# Autodesk Inventor assembly: TuppyMkIV Assembly
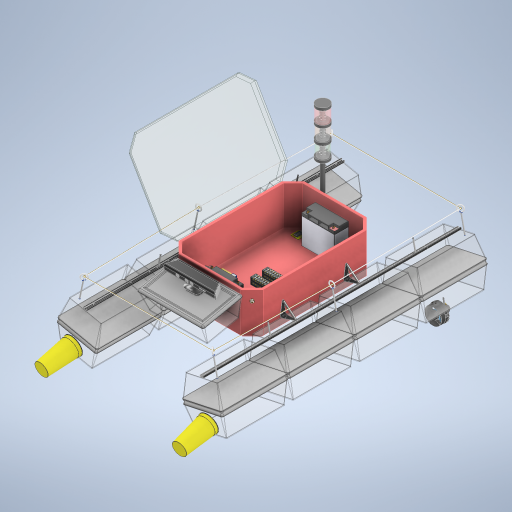
[picture p0: Inventor's stored thumbnail of the model, 512x512]
Saved by Autodesk Inventor 2024 (Build 280153000, 153)
## iProperties
Created: 2023-06-09
Part Number: TuppyMkIV Assembly
Document SubType Name: Assembly
Designer: 18179
Author: 18179
## Documents named in this file (27)
- C:\Users\18179\Desktop\TuppyMkIV\TuppyMkIV Assembly.iam
- C:\Users\18179\Desktop\TuppyMkIV\SmallContainerAssembly.iam
- C:\Users\18179\Desktop\TuppyMkIV\WaterAndBoatLimit.ipt
- C:\Users\18179\Desktop\TuppyMkIV\T200Thruster.ipt
- C:\Users\18179\Desktop\TuppyMkIV\ESC_Assembly.iam
- C:\Users\18179\Desktop\TuppyMkIV\BigContainerLid.ipt
- C:\Users\18179\Desktop\TuppyMkIV\BigContainer.ipt
- C:\Users\18179\Desktop\TuppyMkIV\LightTower.ipt
- C:\Users\18179\Desktop\TuppyMkIV\ProArduino.ipt
- C:\Users\18179\Desktop\TuppyMkIV\RPI\Raspberry Pi 4 Model B.iam
- C:\Users\18179\Downloads\kinect-xbox-360.snapshot.4\Kinect\Kinect.ipt
- C:\Users\18179\Desktop\TuppyMkIV\12Vto5V Converter.ipt
- C:\Users\18179\Desktop\TuppyMkIV\Battery.ipt
- C:\Users\18179\Desktop\TuppyMkIV\CableGland.ipt
- C:\Users\18179\Desktop\TuppyMkIV\RC_Receiver.ipt
- C:\Users\18179\Desktop\TuppyMkIV\EyeBolt.ipt
- C:\Users\18179\Desktop\TuppyMkIV\Hinge.ipt
- C:\Users\18179\Desktop\TuppyMkIV\Hinge_MIR.ipt
- C:\Users\18179\Desktop\TuppyMkIV\Dickey'sBigYellowCup.ipt
- C:\Users\18179\Desktop\TuppyMkIV\C-Channel.ipt
- C:\Users\18179\Desktop\TuppyMkIV\TerminalBlock.ipt
- C:\Users\18179\Desktop\TuppyMkIV\TerminalBlockLid.ipt
- C:\Users\18179\Desktop\TuppyMkIV\Steelbar.ipt
- C:\Users\18179\Desktop\TuppyMkIV\Steelbar_MIR.ipt
- C:\Users\18179\Desktop\TuppyMkIV\C-Channel_7.334in.ipt
- C:\Users\18179\Desktop\TuppyMkIV\TuppyMkIV Assembly\AIP\Cable and Harness\TuppyMkIV Assembly.Harness4.iam
- C:\Users\18179\Desktop\TuppyMkIV\TeeBolt.ipt
## Components (73 placed, 26 different names)
1. WaterAndBoatLimit:1
2. BigContainer:1 — Mate:8, Mate:9, Mate:10, Mate:18, Mate:19, Mate:20, Mate:29, Mate:30, Mate:31, Mate:32, Mate:33, Mate:34, Flush:29, Rotational:1, Mate:36, Mate:37, Mate:38, Mate:39, Mate:45, Mate:51, Mate:52, Mate:53, Mate:54, Mate:55, Mate:56, Mate:57, Flush:36, Flush:37, Mate:58, Mate:59, Mate:60, Mate:63, Mate:64, Flush:45, Mate:75, Mate:76, Angle:1, Angle:2, Angle:3, Mate:98, Mate:103, Mate:104, Mate:105, Mate:106, Mate:107
3. SmallContainerAssembly:1 [sub-assembly] — Flush:1, Flush:4, Flush:5, Mate:1, Flush:13, Flush:14, Mate:81, Mate:82, Tangent:2
4. SmallContainerAssembly:2 [sub-assembly] — Flush:1, Flush:3, Flush:4, Mate:1, Mate:2, Mate:7
5. SmallContainerAssembly:3 [sub-assembly] — Flush:2, Flush:3, Flush:5, Flush:6, Mate:3, Mate:43, Flush:31, Flush:33
6. SmallContainerAssembly:4 [sub-assembly] — Flush:2, Flush:6, Mate:2, Mate:3
7. SmallContainerAssembly:5 [sub-assembly] — Mate:86, Tangent:7, Tangent:8
8. SmallContainerAssembly:6 [sub-assembly] — Mate:7, Mate:8, Mate:10, Mate:66, Flush:43
9. SmallContainerAssembly:7 [sub-assembly] — Flush:13, Flush:14, Mate:84, Tangent:5, Tangent:6, Flush:51, Flush:52, Mate:92
10. SmallContainerAssembly:8 [sub-assembly] — Mate:9, Mate:65, Flush:44, Mate:85, Tangent:13, Tangent:14
11. SmallContainerAssembly:9 [sub-assembly] — Mate:80, Mate:83, Tangent:1
12. SmallContainerAssembly:10 [sub-assembly]
13. SmallContainerAssembly:11 [sub-assembly] — Mate:44, Flush:32, Flush:34
14. SmallContainerAssembly:12 [sub-assembly]
15. SmallContainerAssembly:13 [sub-assembly] — Mate:87, Tangent:9, Tangent:10
16. SmallContainerAssembly:14 [sub-assembly] — Mate:18, Mate:19, Mate:77, Flush:46
17. SmallContainerAssembly:15 [sub-assembly] — Mate:88, Tangent:3, Tangent:4, Mate:93, Flush:53, Flush:54
18. SmallContainerAssembly:16 [sub-assembly] — Mate:20, Mate:78, Mate:79, Mate:89, Tangent:11, Tangent:12
19. ESC_Assembly:1 [sub-assembly] — Mate:29, Mate:31, Mate:33
20. ESC_Assembly:2 [sub-assembly] — Mate:30, Mate:32, Mate:34
21. BigContainerLid:1 — Flush:29, Rotational:1
22. LightTower:1 — Mate:57, Flush:36, Flush:37
23. ProArduino:1 — Mate:36
24. Raspberry Pi 4 Model B:1 [sub-assembly] — Mate:37
25. T200Thruster:1 — Mate:43, Flush:31, Flush:33
26. T200Thruster:2 — Mate:44, Flush:32, Flush:34
27. SmallContainerAssembly:20 [sub-assembly] — Mate:38, Mate:39, Mate:40, Mate:41, Mate:42, Mate:58
28. Kinect:1 — Mate:40, Mate:41, Mate:42
29. 12Vto5V Converter:2 — Mate:45
30. Battery:1 — Mate:104, Mate:106, Flush:56, Flush:59
31. Battery:2 — Mate:105, Mate:107, Flush:55, Mate:108
32. CableGland:1 — Mate:51, Mate:52, Angle:3
33. CableGland:2 — Mate:53, Mate:56, Angle:2
34. CableGland:3 — Mate:54, Mate:55, Angle:1
35. RC_Receiver:1 — Mate:60, Flush:38
36. RC_Receiver:2 — Mate:59, Flush:38
37. Hinge:1 — Mate:63, Mate:69, Mate:70, Mate:109, Mate:111, Mate:112
38. Hinge:2 — Mate:64, Mate:67, Mate:68, Flush:43, Mate:113, Mate:114, Mate:116
39. Hinge:3 — Mate:65, Mate:69, Mate:70, Flush:44, Mate:110
40. Hinge:4 — Mate:66, Mate:67, Mate:68, Mate:115
41. Hinge_MIR:1 — Mate:71, Mate:72, Mate:75, Mate:118, Mate:119, Mate:120
42. Hinge_MIR:2 — Mate:73, Mate:74, Mate:76, Flush:46, Mate:122, Mate:123, Mate:124
43. Hinge_MIR:3 — Mate:71, Mate:72, Mate:78, Mate:79, Mate:117
44. Hinge_MIR:4 — Mate:73, Mate:74, Mate:77, Mate:121
45. Dickey'sBigYellowCup:1 — Mate:81, Mate:82, Tangent:2
46. Dickey'sBigYellowCup:2 — Mate:80, Mate:83, Tangent:1
47. EyeBolt:1 — Mate:88, Tangent:3, Tangent:4
48. EyeBolt:2 — Mate:89, Tangent:11, Tangent:12
49. EyeBolt:3 — Mate:87, Tangent:9, Tangent:10
50. EyeBolt:4 — Mate:86, Tangent:7, Tangent:8
51. EyeBolt:5 — Mate:85, Tangent:13, Tangent:14
52. EyeBolt:6 — Mate:84, Tangent:5, Tangent:6
53. C-Channel:1 — Mate:91, Flush:49, Flush:50, Mate:93, Flush:53, Flush:54, Mate:131, Mate:132, Mate:133, Mate:134
54. C-Channel:2 — Mate:91, Flush:49, Flush:50, Mate:126, Flush:62, Flush:63
55. C-Channel:3 — Mate:90, Flush:47, Flush:48, Flush:51, Flush:52, Mate:92, Mate:127, Mate:128, Mate:129, Mate:130
56. C-Channel:4 — Mate:90, Flush:47, Flush:48, Flush:60, Mate:125, Flush:61
57. TerminalBlock:1 — Mate:94, Mate:95, Mate:96, Mate:97, Flush:58
58. TerminalBlockLid:1 — Mate:94, Mate:95
59. TerminalBlock:2 — Mate:96, Mate:97, Mate:98, Flush:59
60. TerminalBlock:3 — Mate:108, Flush:57
61. TerminalBlockLid:2
62. TerminalBlock:4 — Mate:103
63. Steelbar:1 — Mate:109, Mate:110, Mate:111, Mate:112
64. Steelbar:2 — Mate:113, Mate:114, Mate:115, Mate:116
65. Steelbar_MIR:1 — Mate:117, Mate:118, Mate:119, Mate:120
66. Steelbar_MIR:2 — Mate:121, Mate:122, Mate:123, Mate:124
67. C-Channel_7.334in:1 — Flush:60, Mate:125, Flush:61
68. C-Channel_7.334in:2 — Mate:126, Flush:62, Flush:63
69. Harness4 [sub-assembly]
70. TeeBolt:1 — Mate:131, Mate:132
71. TeeBolt:2 — Mate:133, Mate:134
72. TeeBolt:3 — Mate:129, Mate:130
73. TeeBolt:4 — Mate:127, Mate:128
## Relationships (193: Mate 118, Flush 57, Tangent 14, Angle 3, RevoluteJoint 1)
- Flush:1: SmallContainerAssembly:1 ↔ SmallContainerAssembly:2
- Flush:2: SmallContainerAssembly:3 ↔ SmallContainerAssembly:4
- Flush:3: SmallContainerAssembly:2 ↔ SmallContainerAssembly:3
- Flush:4: SmallContainerAssembly:1 ↔ SmallContainerAssembly:2
- Flush:5: SmallContainerAssembly:1 ↔ SmallContainerAssembly:3
- Flush:6: SmallContainerAssembly:3 ↔ SmallContainerAssembly:4
- Mate:1: SmallContainerAssembly:1 ↔ SmallContainerAssembly:2
- Mate:2: SmallContainerAssembly:2 ↔ SmallContainerAssembly:4
- Mate:3: SmallContainerAssembly:3 ↔ SmallContainerAssembly:4
- [Flush]: SmallContainerAssembly:5 ↔ SmallContainerAssembly:6
- [Flush]: SmallContainerAssembly:7 ↔ SmallContainerAssembly:8
- [Flush]: SmallContainerAssembly:6 ↔ SmallContainerAssembly:7
- [Flush]: SmallContainerAssembly:5 ↔ SmallContainerAssembly:6
- [Flush]: SmallContainerAssembly:5 ↔ SmallContainerAssembly:7
- [Flush]: SmallContainerAssembly:7 ↔ SmallContainerAssembly:8
- [Mate]: SmallContainerAssembly:5 ↔ SmallContainerAssembly:6
- [Mate]: SmallContainerAssembly:6 ↔ SmallContainerAssembly:8
- [Mate]: SmallContainerAssembly:7 ↔ SmallContainerAssembly:8
- Mate:7: SmallContainerAssembly:2 ↔ SmallContainerAssembly:6
- Flush:13: SmallContainerAssembly:1 ↔ SmallContainerAssembly:7
- Flush:14: SmallContainerAssembly:1 ↔ SmallContainerAssembly:7
- Mate:8: BigContainer:1 ↔ SmallContainerAssembly:6
- Mate:9: BigContainer:1 ↔ SmallContainerAssembly:8
- Mate:10 (177.8 mm): BigContainer:1 ↔ SmallContainerAssembly:6
- [Flush]: SmallContainerAssembly:9 ↔ SmallContainerAssembly:10
- [Flush]: SmallContainerAssembly:11 ↔ SmallContainerAssembly:12
- [Flush]: SmallContainerAssembly:10 ↔ SmallContainerAssembly:11
- [Flush]: SmallContainerAssembly:9 ↔ SmallContainerAssembly:10
- [Flush]: SmallContainerAssembly:9 ↔ SmallContainerAssembly:11
- [Flush]: SmallContainerAssembly:11 ↔ SmallContainerAssembly:12
- [Mate]: SmallContainerAssembly:9 ↔ SmallContainerAssembly:10
- [Mate]: SmallContainerAssembly:10 ↔ SmallContainerAssembly:12
- [Mate]: SmallContainerAssembly:11 ↔ SmallContainerAssembly:12
- [Flush]: SmallContainerAssembly:13 ↔ SmallContainerAssembly:14
- [Flush]: SmallContainerAssembly:15 ↔ SmallContainerAssembly:16
- [Flush]: SmallContainerAssembly:14 ↔ SmallContainerAssembly:15
- [Flush]: SmallContainerAssembly:13 ↔ SmallContainerAssembly:14
- [Flush]: SmallContainerAssembly:13 ↔ SmallContainerAssembly:15
- [Flush]: SmallContainerAssembly:15 ↔ SmallContainerAssembly:16
- [Mate]: SmallContainerAssembly:13 ↔ SmallContainerAssembly:14
- [Mate]: SmallContainerAssembly:14 ↔ SmallContainerAssembly:16
- [Mate]: SmallContainerAssembly:15 ↔ SmallContainerAssembly:16
- [Mate]: SmallContainerAssembly:10 ↔ SmallContainerAssembly:14
- [Flush]: SmallContainerAssembly:9 ↔ SmallContainerAssembly:15
- [Flush]: SmallContainerAssembly:9 ↔ SmallContainerAssembly:15
- Mate:18: BigContainer:1 ↔ SmallContainerAssembly:14
- Mate:19 (177.8 mm): BigContainer:1 ↔ SmallContainerAssembly:14
- Mate:20: BigContainer:1 ↔ SmallContainerAssembly:16
- Mate:29: BigContainer:1 ↔ ESC_Assembly:1
- Mate:30: BigContainer:1 ↔ ESC_Assembly:2
- Mate:31 (25.4 mm): BigContainer:1 ↔ ESC_Assembly:1
- Mate:32 (25.4 mm): BigContainer:1 ↔ ESC_Assembly:2
- Mate:33 (50.8 mm): BigContainer:1 ↔ ESC_Assembly:1
- Mate:34 (50.8 mm): BigContainer:1 ↔ ESC_Assembly:2
- Flush:29: BigContainer:1 ↔ BigContainerLid:1
- Rotational:1 [RevoluteJoint]: BigContainer:1 ↔ BigContainerLid:1
- Mate:36: BigContainer:1 ↔ ProArduino:1
- Mate:37 (2.54 mm): BigContainer:1 ↔ Raspberry Pi 4 Model B:1
- Mate:38: BigContainer:1 ↔ SmallContainerAssembly:20
- Mate:39 (12.7 mm): BigContainer:1 ↔ SmallContainerAssembly:20
- Mate:40: SmallContainerAssembly:20 ↔ Kinect:1
- Mate:41 (101.6 mm): SmallContainerAssembly:20 ↔ Kinect:1
- Mate:42 (76.2 mm): SmallContainerAssembly:20 ↔ Kinect:1
- Mate:43: SmallContainerAssembly:3 ↔ T200Thruster:1
- Mate:44: SmallContainerAssembly:11 ↔ T200Thruster:2
- Flush:31 (127 mm): SmallContainerAssembly:3 ↔ T200Thruster:1
- Flush:32 (127 mm): SmallContainerAssembly:11 ↔ T200Thruster:2
- Flush:33 (50.8 mm): SmallContainerAssembly:3 ↔ T200Thruster:1
- Flush:34 (50.8 mm): SmallContainerAssembly:11 ↔ T200Thruster:2
- Mate:45: BigContainer:1 ↔ 12Vto5V Converter:2
- Mate:51: BigContainer:1 ↔ CableGland:1
- Mate:52: BigContainer:1 ↔ CableGland:1
- Mate:53: BigContainer:1 ↔ CableGland:2
- Mate:54: BigContainer:1 ↔ CableGland:3
- Mate:55: BigContainer:1 ↔ CableGland:3
- Mate:56: BigContainer:1 ↔ CableGland:2
- Mate:57: BigContainer:1 ↔ LightTower:1
- Flush:36 (50.8 mm): BigContainer:1 ↔ LightTower:1
- Flush:37 (114.3 mm): BigContainer:1 ↔ LightTower:1
- Mate:58 (-12.7 mm): BigContainer:1 ↔ SmallContainerAssembly:20
- Mate:59: BigContainer:1 ↔ RC_Receiver:2
- Mate:60: BigContainer:1 ↔ RC_Receiver:1
- Flush:38: RC_Receiver:1 ↔ RC_Receiver:2
- Mate:63: BigContainer:1 ↔ Hinge:1
- Mate:64: BigContainer:1 ↔ Hinge:2
- Mate:65: SmallContainerAssembly:8 ↔ Hinge:3
- Mate:66: SmallContainerAssembly:6 ↔ Hinge:4
- Mate:67: Hinge:2 ↔ Hinge:4
- Mate:68: Hinge:2 ↔ Hinge:4
- Mate:69: Hinge:1 ↔ Hinge:3
- Mate:70: Hinge:1 ↔ Hinge:3
- Flush:43 (152.4 mm): SmallContainerAssembly:6 ↔ Hinge:2
- Flush:44 (-152.4 mm): SmallContainerAssembly:8 ↔ Hinge:3
- Flush:45 (-229.87 mm): BigContainer:1
- Mate:71: Hinge_MIR:1 ↔ Hinge_MIR:3
- Mate:72: Hinge_MIR:1 ↔ Hinge_MIR:3
- Mate:73: Hinge_MIR:2 ↔ Hinge_MIR:4
- Mate:74: Hinge_MIR:2 ↔ Hinge_MIR:4
- Mate:75: BigContainer:1 ↔ Hinge_MIR:1
- Mate:76: BigContainer:1 ↔ Hinge_MIR:2
- Mate:77: SmallContainerAssembly:14 ↔ Hinge_MIR:4
- Mate:78: SmallContainerAssembly:16 ↔ Hinge_MIR:3
- Mate:79 (152.4 mm): SmallContainerAssembly:16 ↔ Hinge_MIR:3
- Flush:46 (152.4 mm): SmallContainerAssembly:14 ↔ Hinge_MIR:2
- Mate:80: SmallContainerAssembly:9 ↔ Dickey'sBigYellowCup:2
- Mate:81: SmallContainerAssembly:1 ↔ Dickey'sBigYellowCup:1
- Mate:82 (-76.2 mm): SmallContainerAssembly:1 ↔ Dickey'sBigYellowCup:1
- Mate:83 (-76.2 mm): SmallContainerAssembly:9 ↔ Dickey'sBigYellowCup:2
- Tangent:1 (6.35 mm): SmallContainerAssembly:9 ↔ Dickey'sBigYellowCup:2
- Tangent:2 (6.35 mm): SmallContainerAssembly:1 ↔ Dickey'sBigYellowCup:1
- Mate:84: SmallContainerAssembly:7 ↔ EyeBolt:6
- Mate:85: SmallContainerAssembly:8 ↔ EyeBolt:5
- Mate:86: SmallContainerAssembly:5 ↔ EyeBolt:4
- Mate:87: SmallContainerAssembly:13 ↔ EyeBolt:3
- Mate:88: SmallContainerAssembly:15 ↔ EyeBolt:1
- Mate:89: SmallContainerAssembly:16 ↔ EyeBolt:2
- Tangent:3 (25.4 mm): SmallContainerAssembly:15 ↔ EyeBolt:1
- Tangent:4 (25.4 mm): SmallContainerAssembly:15 ↔ EyeBolt:1
- Tangent:5 (25.4 mm): SmallContainerAssembly:7 ↔ EyeBolt:6
- Tangent:6 (25.4 mm): SmallContainerAssembly:7 ↔ EyeBolt:6
- Tangent:7 (25.4 mm): SmallContainerAssembly:5 ↔ EyeBolt:4
- Tangent:8 (25.4 mm): SmallContainerAssembly:5 ↔ EyeBolt:4
- Tangent:9 (25.4 mm): SmallContainerAssembly:13 ↔ EyeBolt:3
- Tangent:10 (25.4 mm): SmallContainerAssembly:13 ↔ EyeBolt:3
- Tangent:11 (12.7 mm): SmallContainerAssembly:16 ↔ EyeBolt:2
- Tangent:12 (12.7 mm): SmallContainerAssembly:16 ↔ EyeBolt:2
- Tangent:13 (12.7 mm): SmallContainerAssembly:8 ↔ EyeBolt:5
- Tangent:14 (12.7 mm): SmallContainerAssembly:8 ↔ EyeBolt:5
- Mate:90: C-Channel:3 ↔ C-Channel:4
- Flush:47: C-Channel:3 ↔ C-Channel:4
- Flush:48: C-Channel:3 ↔ C-Channel:4
- Mate:91: C-Channel:1 ↔ C-Channel:2
- Flush:49: C-Channel:1 ↔ C-Channel:2
- Flush:50: C-Channel:1 ↔ C-Channel:2
- Flush:51 (76.2 mm): SmallContainerAssembly:7 ↔ C-Channel:3
- Flush:52: SmallContainerAssembly:7 ↔ C-Channel:3
- Mate:92: SmallContainerAssembly:7 ↔ C-Channel:3
- Mate:93: SmallContainerAssembly:15 ↔ C-Channel:1
- Flush:53: SmallContainerAssembly:15 ↔ C-Channel:1
- Flush:54 (76.2 mm): SmallContainerAssembly:15 ↔ C-Channel:1
- Angle:1 (43.19 deg): BigContainer:1 ↔ CableGland:3
- Angle:2 (60 deg): BigContainer:1 ↔ CableGland:2
- Angle:3 (45.84 deg): BigContainer:1 ↔ CableGland:1
- Mate:94: TerminalBlock:1 ↔ TerminalBlockLid:1
- Mate:95: TerminalBlock:1 ↔ TerminalBlockLid:1
- Mate:96: TerminalBlock:1 ↔ TerminalBlock:2
- Mate:97: TerminalBlock:1 ↔ TerminalBlock:2
- Mate:98: BigContainer:1 ↔ TerminalBlock:2
- [Mate]: TerminalBlock:3 ↔ TerminalBlockLid:2
- [Mate]: TerminalBlock:3 ↔ TerminalBlockLid:2
- [Mate]: TerminalBlock:3 ↔ TerminalBlock:4
- [Mate]: TerminalBlock:3 ↔ TerminalBlock:4
- Mate:103: BigContainer:1 ↔ TerminalBlock:4
- Mate:104 (5.08 mm): BigContainer:1 ↔ Battery:1
- Mate:105 (5.08 mm): BigContainer:1 ↔ Battery:2
- Mate:106: BigContainer:1 ↔ Battery:1
- Mate:107: BigContainer:1 ↔ Battery:2
- Flush:55 (90.17 mm): Battery:2
- Flush:56 (90.17 mm): Battery:1
- Mate:108 (228.6 mm): Battery:2 ↔ TerminalBlock:3
- Flush:57 (-45.72 mm): TerminalBlock:3
- Flush:58 (-45.72 mm): TerminalBlock:1
- Flush:59 (203.2 mm): Battery:1 ↔ TerminalBlock:2
- Mate:109: Hinge:1 ↔ Steelbar:1
- Mate:110: Hinge:3 ↔ Steelbar:1
- Mate:111: Hinge:1 ↔ Steelbar:1
- Mate:112 (1.016 mm): Hinge:1 ↔ Steelbar:1
- Mate:113: Hinge:2 ↔ Steelbar:2
- Mate:114: Hinge:2 ↔ Steelbar:2
- Mate:115: Hinge:4 ↔ Steelbar:2
- Mate:116 (1.016 mm): Hinge:2 ↔ Steelbar:2
- Mate:117: Hinge_MIR:3 ↔ Steelbar_MIR:1
- Mate:118: Hinge_MIR:1 ↔ Steelbar_MIR:1
- Mate:119: Hinge_MIR:1 ↔ Steelbar_MIR:1
- Mate:120 (1.016 mm): Hinge_MIR:1 ↔ Steelbar_MIR:1
- Mate:121: Hinge_MIR:4 ↔ Steelbar_MIR:2
- Mate:122: Hinge_MIR:2 ↔ Steelbar_MIR:2
- Mate:123: Hinge_MIR:2 ↔ Steelbar_MIR:2
- Mate:124 (1.016 mm): Hinge_MIR:2 ↔ Steelbar_MIR:2
- Flush:60: C-Channel:4 ↔ C-Channel_7.334in:1
- Mate:125: C-Channel:4 ↔ C-Channel_7.334in:1
- Flush:61: C-Channel:4 ↔ C-Channel_7.334in:1
- Mate:126: C-Channel:2 ↔ C-Channel_7.334in:2
- Flush:62: C-Channel:2 ↔ C-Channel_7.334in:2
- Flush:63: C-Channel:2 ↔ C-Channel_7.334in:2
- Mate:127: C-Channel:3 ↔ TeeBolt:4
- Mate:128: C-Channel:3 ↔ TeeBolt:4
- Mate:129: C-Channel:3 ↔ TeeBolt:3
- Mate:130: C-Channel:3 ↔ TeeBolt:3
- Mate:131: C-Channel:1 ↔ TeeBolt:1
- Mate:132: C-Channel:1 ↔ TeeBolt:1
- Mate:133: C-Channel:1 ↔ TeeBolt:2
- Mate:134: C-Channel:1 ↔ TeeBolt:2
## Named parameters: d126_d117 = 0 mm, d127_d118 = 0 mm, d128_d119 = 0 mm, d129_d120 = 0 mm, d130_d121 = 0 mm, d131_d122 = 0 mm, d132_d123 = 0 mm, d133_d124 = 0 mm, d134_d125 = 0 mm, d141_d135 = 0 mm, d142_d136 = 0 mm, d143_d137 = 0 mm, d144_d117 = 0 mm, d145_d118 = 0 mm, d146_d119 = 0 mm, d147_d120 = 0 mm, d148_d121 = 0 mm, d149_d122 = 0 mm, d150_d123 = 0 mm, d151_d124 = 0 mm, d152_d125 = 0 mm, d153_d126_d117 = 0 mm, d154_d127_d118 = 0 mm, d155_d128_d119 = 0 mm, d156_d129_d120 = 0 mm, d157_d130_d121 = 0 mm, d158_d131_d122 = 0 mm, d159_d132_d123 = 0 mm, d160_d133_d124 = 0 mm, d161_d134_d125 = 0 mm, d313_d308 = 0 mm, d314_d309 = 0 mm, d315_d310 = 0 mm, d316_d311 = 0 mm, Finish1_Area = 3440.14, Finish2_Area = 144.689, Finish3_Area = 144.689, Finish4_Area = 6519.08
note: some values were not read from the file. Shown as the stored number, unit unknown: "Finish1_Area", "Finish2_Area", "Finish3_Area", "Finish4_Area".
